# Autodesk Inventor assembly: SAR330  x 5 left + limit switches
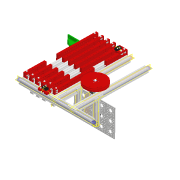
[picture p0: Inventor's stored thumbnail of the model, 180x180]
Saved by Autodesk Inventor 2020 (Build 240168000, 168)
## iProperties
Created: 2019-11-17
Part Number: SAR330  x 5 left + limit switches
Document SubType Name: Assembly
Designer: ball
Author: ball
## Documents named in this file (21)
- C:\FTC\FTC8863CAD\2019 Robot\Delivery\SAR330  x 5 left + limit switches.iam
- C:\FTC\FTC8863CAD\Actobotics\605 parts\605630.ipt
- C:\FTC\FTC8863CAD\StepLibraries\Nuts\2-56 NYLON-INSERT LOCKNUT.ipt
- C:\FTC\FTC8863CAD\StepLibraries\Screws\M3 x 25 HEX HEAD CAP SCREW.ipt
- C:\FTC\FTC8863CAD\2019 Robot\Delivery\Limit switch trigger spacer.ipt
- C:\FTC\FTC8863CAD\Actobotics\565 parts\565046.ipt
- C:\FTC\FTC8863CAD\Actobotics\585 parts\585075.ipt
- C:\FTC\FTC8863CAD\Actobotics\565 parts\xrail_3.5in.ipt
- C:\FTC\FTC8863CAD\Andymark\am-3461a NeveRest 4 with Motor REV3.ipt
- C:\FTC\FTC8863CAD\Actobotics\555 parts\555116 assembly.ipt
- C:\FTC\FTC8863CAD\2019 Robot\Delivery\double_spool_6mm_clamping_hubAssembly.iam
- C:\FTC\FTC8863CAD\2019 Robot\Generic Parts\limit switch mount to xrail.ipt
- C:\FTC\FTC8863CAD\StepLibraries\Screws\2-56x.5_18-8 SS PAN HEAD PHILLIPS MACHINE SCREW.ipt
- C:\FTC\FTC8863CAD\StepLibraries\Screws\6-32x.375_18-8 SS TRUSS HEAD PHILLIPS MACHINE SCREW.ipt
- C:\FTC\FTC8863CAD\2019 Robot\Delivery\Limit switch top + mount.iam
- C:\FTC\FTC8863CAD\Actobotics\585 parts\585002.ipt
- C:\FTC\FTC8863CAD\2019 Robot\Delivery\Coupler lift long left bracket + pulleys.iam
- C:\FTC\FTC8863CAD\2019 Robot\Delivery\SAR330  x 5 + couplers left.iam
- C:\FTC\FTC8863CAD\2019 Robot\Delivery\Coupler lift short left + pulleys.iam
- C:\FTC\FTC8863CAD\2019 Robot\Delivery\support.ipt
- C:\FTC\FTC8863CAD\2019 Robot\Delivery\Lift mount insert left.ipt
## Components (29 placed, 20 different names)
1. SAR330  x 5 + couplers left:1 [sub-assembly] — Mate:5, Flush:7, Mate:18, Mate:19, Mate:33, Mate:34, Mate:35, Mate:36, Flush:16, Mate:38, Flush:20, Mate:40, Flush:21, Flush:24, Mate:43, Flush:34, Flush:35, Mate:68, Mate:70, Mate:72, Mate:73, Mate:74, Flush:36
2. 605630:2 — Mate:5, Flush:7, Flush:33, Mate:61, Mate:63, Mate:64, Mate:65
3. M3 x 25 HEX HEAD CAP SCREW:1 — Mate:18, Mate:19, Mate:25, Mate:26
4. Limit switch trigger spacer:1 — Mate:25, Mate:26
5. M3 x 25 HEX HEAD CAP SCREW:2 — Mate:33
6. M3 x 25 HEX HEAD CAP SCREW:3 — Mate:34
7. Coupler lift short left + pulleys:1 [sub-assembly] — Mate:35, Mate:36, Flush:16, Flush:17, Flush:19, Mate:37
8. 565046:1 — Flush:17, Flush:19, Mate:37, Mate:39, Flush:22, Mate:42, Flush:25, Mate:48, Mate:49, Mate:60, Flush:32, Mate:75, Flush:37
9. 585075:1 — Mate:38, Flush:20, Mate:39
10. xrail_3.5in:1 — Mate:40, Flush:21, Flush:22, Mate:41, Flush:23, Flush:27, Symmetry:1, Flush:29, Mate:71
11. 585075:2 — Mate:41, Flush:23, Flush:24
12. 565046:2 — Mate:42, Flush:25, Mate:43, Mate:44, Flush:26, Mate:46, Flush:28, Mate:50, Mate:51
13. xrail_3.5in:2 — Mate:44, Flush:26, Flush:27, Mate:45, Mate:47, Mate:52, Symmetry:1, Mate:56, Mate:57, Mate:69
14. 585075:3 — Mate:45, Mate:46, Mate:47
15. 585075:4 — Mate:48, Flush:28, Mate:49
16. 585075:5 — Mate:50, Mate:51, Mate:52
17. am-3461a NeveRest 4 with Motor REV3:1 — Mate:53, Flush:29, Mate:54, Mate:55, Flush:30, Flush:31, Mate:58, Mate:59
18. 555116 assembly:1 — Mate:54, Flush:31
19. 555116 assembly:2 — Mate:55, Flush:30, Mate:56, Mate:57
20. double_spool_6mm_clamping_hubAssembly:1 [sub-assembly] — Mate:58, Mate:59
21. limit switch mount to xrail:1 — Mate:60, Flush:32, Flush:33, Mate:61, Mate:62, Angle:1, Mate:66, Mate:67
22. 2-56 NYLON-INSERT LOCKNUT:4 — Mate:62, Mate:63, Angle:1
23. 2-56x.5_18-8 SS PAN HEAD PHILLIPS MACHINE SCREW:1 — Mate:64, Mate:65
24. 6-32x.375_18-8 SS TRUSS HEAD PHILLIPS MACHINE SCREW:1 — Mate:66, Mate:67
25. Limit switch top + mount:1 [sub-assembly] — Flush:34, Flush:35, Mate:68
26. 585002:1 — Mate:69, Mate:70, Mate:71
27. Coupler lift long left bracket + pulleys:1 [sub-assembly] — Mate:72, Mate:73, Mate:74, Flush:39
28. Lift mount insert left:1 — Mate:75, Flush:36, Flush:37
29. support:1 — Flush:39
## Relationships (73: Mate 48, Flush 23, Symmetry 1, Angle 1)
- Mate:5 (1.27 mm): SAR330  x 5 + couplers left:1 ↔ 605630:2
- Flush:7: SAR330  x 5 + couplers left:1 ↔ 605630:2
- Mate:18: SAR330  x 5 + couplers left:1 ↔ M3 x 25 HEX HEAD CAP SCREW:1
- Mate:19 (6 mm): SAR330  x 5 + couplers left:1 ↔ M3 x 25 HEX HEAD CAP SCREW:1
- Mate:25: M3 x 25 HEX HEAD CAP SCREW:1 ↔ Limit switch trigger spacer:1
- Mate:26: M3 x 25 HEX HEAD CAP SCREW:1 ↔ Limit switch trigger spacer:1
- Mate:33: SAR330  x 5 + couplers left:1 ↔ M3 x 25 HEX HEAD CAP SCREW:2
- Mate:34: SAR330  x 5 + couplers left:1 ↔ M3 x 25 HEX HEAD CAP SCREW:3
- Mate:35: SAR330  x 5 + couplers left:1 ↔ Coupler lift short left + pulleys:1
- Mate:36: SAR330  x 5 + couplers left:1 ↔ Coupler lift short left + pulleys:1
- Flush:16: SAR330  x 5 + couplers left:1 ↔ Coupler lift short left + pulleys:1
- Flush:17: Coupler lift short left + pulleys:1 ↔ 565046:1
- Flush:19: Coupler lift short left + pulleys:1 ↔ 565046:1
- Mate:37: Coupler lift short left + pulleys:1 ↔ 565046:1
- Mate:38: SAR330  x 5 + couplers left:1 ↔ 585075:1
- Flush:20: SAR330  x 5 + couplers left:1 ↔ 585075:1
- Mate:39: 565046:1 ↔ 585075:1
- Mate:40: SAR330  x 5 + couplers left:1 ↔ xrail_3.5in:1
- Flush:21: SAR330  x 5 + couplers left:1 ↔ xrail_3.5in:1
- Flush:22 (100.2792 mm): 565046:1 ↔ xrail_3.5in:1
- Mate:41: xrail_3.5in:1 ↔ 585075:2
- Flush:23: xrail_3.5in:1 ↔ 585075:2
- Flush:24: SAR330  x 5 + couplers left:1 ↔ 585075:2
- Mate:42: 565046:1 ↔ 565046:2
- Flush:25: 565046:1 ↔ 565046:2
- Mate:43 (57.15 mm): SAR330  x 5 + couplers left:1 ↔ 565046:2
- Mate:44: 565046:2 ↔ xrail_3.5in:2
- Flush:26: 565046:2 ↔ xrail_3.5in:2
- Flush:27: xrail_3.5in:1 ↔ xrail_3.5in:2
- Mate:45: xrail_3.5in:2 ↔ 585075:3
- Mate:46: 565046:2 ↔ 585075:3
- Mate:47: xrail_3.5in:2 ↔ 585075:3
- Mate:48: 565046:1 ↔ 585075:4
- Flush:28: 565046:2 ↔ 585075:4
- Mate:49: 565046:1 ↔ 585075:4
- Mate:50: 565046:2 ↔ 585075:5
- Mate:51: 565046:2 ↔ 585075:5
- Mate:52: xrail_3.5in:2 ↔ 585075:5
- Symmetry:1: xrail_3.5in:1 ↔ xrail_3.5in:2
- Mate:53: am-3461a NeveRest 4 with Motor REV3:1
- Flush:29: xrail_3.5in:1 ↔ am-3461a NeveRest 4 with Motor REV3:1
- Mate:54: am-3461a NeveRest 4 with Motor REV3:1 ↔ 555116 assembly:1
- Mate:55: am-3461a NeveRest 4 with Motor REV3:1 ↔ 555116 assembly:2
- Flush:30 (19.05 mm): am-3461a NeveRest 4 with Motor REV3:1 ↔ 555116 assembly:2
- Flush:31 (22.86 mm): am-3461a NeveRest 4 with Motor REV3:1 ↔ 555116 assembly:1
- Mate:56: xrail_3.5in:2 ↔ 555116 assembly:2
- Mate:57: xrail_3.5in:2 ↔ 555116 assembly:2
- Mate:58: am-3461a NeveRest 4 with Motor REV3:1 ↔ double_spool_6mm_clamping_hubAssembly:1
- Mate:59: am-3461a NeveRest 4 with Motor REV3:1 ↔ double_spool_6mm_clamping_hubAssembly:1
- Mate:60: 565046:1 ↔ limit switch mount to xrail:1
- Flush:32: 565046:1 ↔ limit switch mount to xrail:1
- Flush:33: 605630:2 ↔ limit switch mount to xrail:1
- Mate:61: 605630:2 ↔ limit switch mount to xrail:1
- Mate:62: limit switch mount to xrail:1 ↔ 2-56 NYLON-INSERT LOCKNUT:4
- Mate:63: 605630:2 ↔ 2-56 NYLON-INSERT LOCKNUT:4
- Angle:1 (0 deg): limit switch mount to xrail:1 ↔ 2-56 NYLON-INSERT LOCKNUT:4
- Mate:64: 605630:2 ↔ 2-56x.5_18-8 SS PAN HEAD PHILLIPS MACHINE SCREW:1
- Mate:65: 605630:2 ↔ 2-56x.5_18-8 SS PAN HEAD PHILLIPS MACHINE SCREW:1
- Mate:66: limit switch mount to xrail:1 ↔ 6-32x.375_18-8 SS TRUSS HEAD PHILLIPS MACHINE SCREW:1
- Mate:67: limit switch mount to xrail:1 ↔ 6-32x.375_18-8 SS TRUSS HEAD PHILLIPS MACHINE SCREW:1
- Flush:34: SAR330  x 5 + couplers left:1 ↔ Limit switch top + mount:1
- Flush:35 (2.54 mm): SAR330  x 5 + couplers left:1 ↔ Limit switch top + mount:1
- Mate:68: SAR330  x 5 + couplers left:1 ↔ Limit switch top + mount:1
- Mate:69: xrail_3.5in:2 ↔ 585002:1
- Mate:70: SAR330  x 5 + couplers left:1 ↔ 585002:1
- Mate:71: xrail_3.5in:1 ↔ 585002:1
- Mate:72: SAR330  x 5 + couplers left:1 ↔ Coupler lift long left bracket + pulleys:1
- Mate:73: SAR330  x 5 + couplers left:1 ↔ Coupler lift long left bracket + pulleys:1
- Mate:74: SAR330  x 5 + couplers left:1 ↔ Coupler lift long left bracket + pulleys:1
- Mate:75: 565046:1 ↔ Lift mount insert left:1
- Flush:36: SAR330  x 5 + couplers left:1 ↔ Lift mount insert left:1
- Flush:37: 565046:1 ↔ Lift mount insert left:1
- Flush:39: Coupler lift long left bracket + pulleys:1 ↔ support:1
